# Autodesk Inventor assembly: IK_test
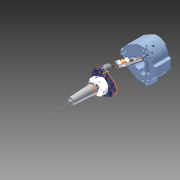
[picture p0: Inventor's stored thumbnail of the model, 180x180]
Saved by Autodesk Inventor 2011 SP2 (Build 150309200, 309)
## iProperties
Created: 2013-03-14
Part Number: IK_test
Document SubType Name: Assembly
Designer: sungwook
Author: sungwook
## Documents named in this file (6)
- C:\Users\sungwook\Documents\Inventor\Micron22_top_adj_02082013\Assembly\IK_test.iam
- C:\Users\sungwook\Documents\Inventor\Micron22_top_adj_02082013\Parts\Main\Platform_Top_14mm_Rev.ipt
- C:\Users\sungwook\Documents\Inventor\Micron22_top_adj_02082013\Parts\Main\Platform_Base_20mm_Rev2.ipt
- C:\Users\sungwook\Documents\Inventor\Micron22_top_adj_02082013\Parts\Tool\ASM_Tool_Tip_Rev.iam
- C:\Users\sungwook\Documents\Inventor\Micron22_top_adj_02082013\Assembly\ASM_Motor_Unit_Part1_Rev.iam
- C:\Users\sungwook\Documents\Inventor\Micron22_top_adj_02082013\Assembly\ASM_Motor_Unit_Part2_Rev.iam
## Components (5 placed, 5 different names)
1. Platform_Top_14mm_Rev:1 — Mate:4, Mate:5, Mate:10, Mate:15
2. Platform_Base_20mm_Rev2:1 — Mate:7, Mate:8, Mate:9, Mate:11, Mate:12, Mate:13, Mate:16
3. ASM_Tool_Tip_Rev:1 [sub-assembly] — Mate:4, Mate:5, Mate:10, Mate:7, Mate:8, Mate:9, Mate:11, Mate:12, Mate:13
4. ASM_Motor_Unit_Part1_Rev:1 [sub-assembly] — Mate:14, Mate:16, Mate:17, Mate:18
5. ASM_Motor_Unit_Part2_Rev:1 [sub-assembly] — Mate:14, Mate:15, Mate:17, Mate:18
## Relationships (14: Mate 14)
- Mate:4: Platform_Top_14mm_Rev:1 ↔ ASM_Tool_Tip_Rev:1
- Mate:5: Platform_Top_14mm_Rev:1 ↔ ASM_Tool_Tip_Rev:1
- Mate:10: Platform_Top_14mm_Rev:1 ↔ ASM_Tool_Tip_Rev:1
- Mate:7 (46 mm): Platform_Base_20mm_Rev2:1 ↔ ASM_Tool_Tip_Rev:1
- Mate:8: Platform_Base_20mm_Rev2:1 ↔ ASM_Tool_Tip_Rev:1
- Mate:9: Platform_Base_20mm_Rev2:1 ↔ ASM_Tool_Tip_Rev:1
- Mate:11 (2 mm): Platform_Base_20mm_Rev2:1 ↔ ASM_Tool_Tip_Rev:1
- Mate:12 (2 mm): Platform_Base_20mm_Rev2:1 ↔ ASM_Tool_Tip_Rev:1
- Mate:13 (80 mm): Platform_Base_20mm_Rev2:1 ↔ ASM_Tool_Tip_Rev:1
- Mate:14: ASM_Motor_Unit_Part1_Rev:1 ↔ ASM_Motor_Unit_Part2_Rev:1
- Mate:15: Platform_Top_14mm_Rev:1 ↔ ASM_Motor_Unit_Part2_Rev:1
- Mate:16: Platform_Base_20mm_Rev2:1 ↔ ASM_Motor_Unit_Part1_Rev:1
- Mate:17: ASM_Motor_Unit_Part1_Rev:1 ↔ ASM_Motor_Unit_Part2_Rev:1
- Mate:18: ASM_Motor_Unit_Part1_Rev:1 ↔ ASM_Motor_Unit_Part2_Rev:1
